# Autodesk Inventor assembly: selection system 2
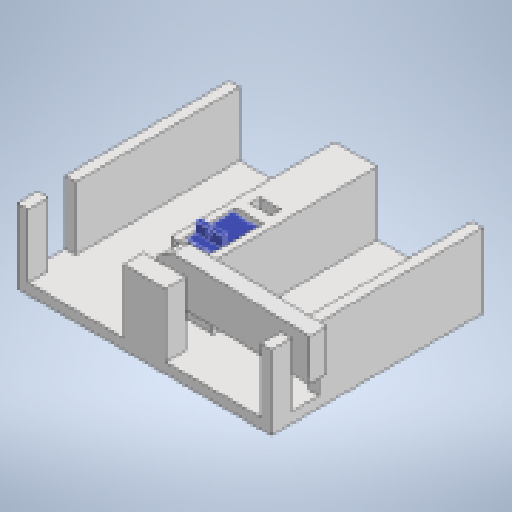
[picture p0: Inventor's stored thumbnail of the model, 512x512]
Saved by Autodesk Inventor 2025.3 (Build 293356000, 356)
## iProperties
Created: 2026-04-13
Part Number: selection system 2
Document SubType Name: Assembly
Designer: kamal
Author: kamal
## Documents named in this file (5)
- C:\Users\kamal\OneDrive\Desktop\Personal\semester 4\Basics of Mechatronics\Full Assembly\selection system 2.iam
- C:\Users\kamal\OneDrive\Desktop\Personal\semester 4\Basics of Mechatronics\Full Assembly\Selection Body V1.ipt
- C:\Users\kamal\OneDrive\Desktop\Personal\semester 4\Basics of Mechatronics\Full Assembly\SG90_Model_A.ipt
- C:\Users\kamal\OneDrive\Desktop\Personal\semester 4\Basics of Mechatronics\Full Assembly\SG90_Arm_Original.ipt
- C:\Users\kamal\OneDrive\Desktop\Personal\semester 4\Basics of Mechatronics\Full Assembly\Servo_Shaft_select_V2.ipt
## Components (4 placed, 4 different names)
1. Selection Body V1:1 — Mate:1, Mate:2, Mate:3
2. SG90_Model_A:1 — Mate:1, Mate:2, Mate:3, Insert:1
3. SG90_Arm_Original:1 — Insert:1, Mate:4, Mate:5, Mate:6
4. Servo_Shaft_select_V2:1 — Mate:4, Mate:5, Mate:6
## Relationships (7: Mate 6, Insert 1)
- Mate:1: Selection Body V1:1 ↔ SG90_Model_A:1
- Mate:2: Selection Body V1:1 ↔ SG90_Model_A:1
- Mate:3: Selection Body V1:1 ↔ SG90_Model_A:1
- Insert:1: SG90_Model_A:1 ↔ SG90_Arm_Original:1
- Mate:4: SG90_Arm_Original:1 ↔ Servo_Shaft_select_V2:1
- Mate:5: SG90_Arm_Original:1 ↔ Servo_Shaft_select_V2:1
- Mate:6: SG90_Arm_Original:1 ↔ Servo_Shaft_select_V2:1
